# Autodesk Inventor assembly: L22ED01D
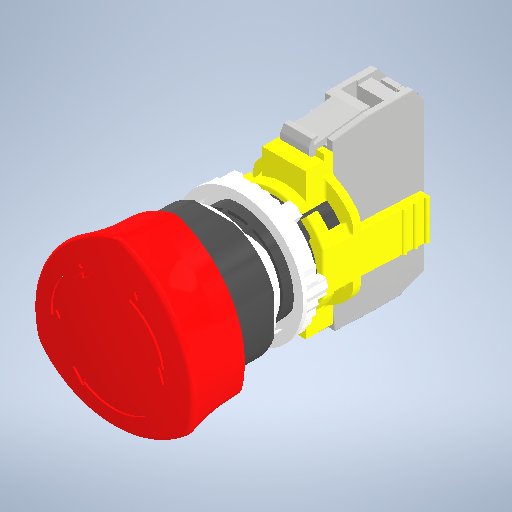
[picture p0: Inventor's stored thumbnail of the model, 512x512]
Saved by Autodesk Inventor 2025.3 (Build 293356000, 356)
## iProperties
Company: Legrand SA
Created: 2008-01-18
Part Number: L22ED01D
Description: STEP AP214
Document SubType Name: Assembly
Designer: louis
Sending System: TRANSCAD
Preprocessor: XStep 1.0
Title: C:/convcao/utilisateur/sortie/fabien.fantini@legrand.fr/21/L22ED01D.stp
## Documents named in this file (19)
- C:\Users\louis\OneDrive\Desktop\R_Trident\02_CAD\01_Standard_Parts\04_ELE_Electrical_Automation\L22ED01D\L22ED01D.iam
- C:\Users\louis\OneDrive\Desktop\R_Trident\02_CAD\01_Standard_Parts\ImportTemp\L22ED01D\L22ED01D\L22ED01D\Part1_Corps principal ( 074228000 - wsp _MASTER -  )_Solide.1 (  de JELE 20955 _ issu de 074228000 - wsp .ipt
- C:\Users\louis\OneDrive\Desktop\R_Trident\02_CAD\01_Standard_Parts\ImportTemp\L22ED01D\L22ED01D\L22ED01D\Part1_Corps de pièce.2 ( _SOL3 - wsp _MASTER -  -Non Smart-  )_Solide.2 (  de JELE 11302 _ issu de _SOL3 .ipt
- C:\Users\louis\OneDrive\Desktop\R_Trident\02_CAD\01_Standard_Parts\ImportTemp\L22ED01D\L22ED01D\L22ED01D\Part1_Corps de pièce.3 ( _SOL4 - wsp _MASTER -  )_Solide.3 (  de JELE 25154 _ issu de _SOL4 - wsp _MASTER.ipt
- C:\Users\louis\OneDrive\Desktop\R_Trident\02_CAD\01_Standard_Parts\ImportTemp\L22ED01D\L22ED01D\L22ED01D\Part1_Corps de pièce.4 ( _SOL5 - wsp _MASTER -  )_Solide.4 (  de JELE 29157 _ issu de _SOL5 - wsp _MASTER.ipt
- C:\Users\louis\OneDrive\Desktop\R_Trident\02_CAD\01_Standard_Parts\ImportTemp\L22ED01D\L22ED01D\L22ED01D\Part1_Corps de pièce.5 ( 075121000 - wsp _MASTER -  )_Solide.5 (  de JELE 40425 _ issu de 075121000 - wsp.ipt
- C:\Users\louis\OneDrive\Desktop\R_Trident\02_CAD\01_Standard_Parts\ImportTemp\L22ED01D\L22ED01D\L22ED01D\Part1_Corps de pièce.6 ( _SOL7 - wsp _MASTER -  )_Solide.6 (  de JELE 41156 _ issu de _SOL7 - wsp _MASTER.ipt
- C:\Users\louis\OneDrive\Desktop\R_Trident\02_CAD\01_Standard_Parts\ImportTemp\L22ED01D\L22ED01D\L22ED01D\Part1_Corps de pièce.7 ( _SOL8 - wsp _MASTER -  )_Solide.7 (  de JELE 64956 _ issu de _SOL8 - wsp _MASTER.ipt
- C:\Users\louis\OneDrive\Desktop\R_Trident\02_CAD\01_Standard_Parts\ImportTemp\L22ED01D\L22ED01D\L22ED01D\Part1_Corps de pièce.8 ( _SOL9 - wsp _MASTER -  -Non Smart-  )_Solide.8 (  de JELE 110028 _ issu de _SOL9.ipt
- C:\Users\louis\OneDrive\Desktop\R_Trident\02_CAD\01_Standard_Parts\ImportTemp\L22ED01D\L22ED01D\L22ED01D\Part1_Corps de pièce.9 ( _SOL10 - wsp _MASTER -  )_Solide.9 (  de JELE 54590 _ issu de _SOL10 - wsp _MAST.ipt
- C:\Users\louis\OneDrive\Desktop\R_Trident\02_CAD\01_Standard_Parts\ImportTemp\L22ED01D\L22ED01D\L22ED01D\Part1_Corps de pièce.10 ( _SOL11 - wsp _MASTER -  -Non Smart-  )_Solide.10 (  de JELE 63513 _ issu de _SO.ipt
- C:\Users\louis\OneDrive\Desktop\R_Trident\02_CAD\01_Standard_Parts\ImportTemp\L22ED01D\L22ED01D\L22ED01D\Part1_Corps de pièce.11 ( _SOL12 - wsp _MASTER -  -Non Smart-  )_Solide.11 (  de JELE 64772 _ issu de _SO.ipt
- C:\Users\louis\OneDrive\Desktop\R_Trident\02_CAD\01_Standard_Parts\ImportTemp\L22ED01D\L22ED01D\L22ED01D\Part1_Corps de pièce.12 ( _SOL13 - wsp _MASTER -  )_Solide.12 (  de JELE 45820 _ issu de _SOL13 - wsp _MA.ipt
- C:\Users\louis\OneDrive\Desktop\R_Trident\02_CAD\01_Standard_Parts\ImportTemp\L22ED01D\L22ED01D\L22ED01D\Part1_Corps de pièce.13 ( _SOL14 - wsp _MASTER -  )_Solide.13 (  de JELE 88964 _ issu de _SOL14 - wsp _MA.ipt
- C:\Users\louis\OneDrive\Desktop\R_Trident\02_CAD\01_Standard_Parts\ImportTemp\L22ED01D\L22ED01D\L22ED01D\Part1_Corps de pièce.14 ( _SOL15 - wsp _MASTER -  )_Solide.14 (  de JELE 108439 _ issu de _SOL15 - wsp _M.ipt
- C:\Users\louis\OneDrive\Desktop\R_Trident\02_CAD\01_Standard_Parts\ImportTemp\L22ED01D\L22ED01D\L22ED01D\Part1_Corps de pièce.15 ( _SOL16 - wsp _MASTER -  -Non Smart-  )_Solide.15 (  de JELE 109844 _ issu de _S.ipt
- C:\Users\louis\OneDrive\Desktop\R_Trident\02_CAD\01_Standard_Parts\ImportTemp\L22ED01D\L22ED01D\L22ED01D\Part1_Corps de pièce.16 ( _SOL17 - wsp _MASTER -  -Non Smart-  )_Solide.16 (  de JELE 110465 _ issu de _S.ipt
- C:\Users\louis\OneDrive\Desktop\R_Trident\02_CAD\01_Standard_Parts\ImportTemp\L22ED01D\L22ED01D\L22ED01D\Part1_Corps de pièce.17 ( _SOL18 - wsp _MASTER -  -Non Smart-  )_Assemble.1.ipt
- C:\Users\louis\OneDrive\Desktop\R_Trident\02_CAD\01_Standard_Parts\ImportTemp\L22ED01D\L22ED01D\L22ED01D\Part1_Corps de pièce.17 ( _SOL18 - wsp _MASTER -  -Non Smart-  )_Assemble.1_1.ipt
## Components (18 placed, 18 different names)
1. Part1_Corps principal ( 074228000 - wsp _MASTER -  )_Solide.1 (  de JELE 20955 _ issu de 074228000 - wsp — Insert:1
2. Part1_Corps de pièce.2 ( _SOL3 - wsp _MASTER -  -Non Smart-  )_Solide.2 (  de JELE 11302 _ issu de _SOL3 — Insert:1
3. Part1_Corps de pièce.3 ( _SOL4 - wsp _MASTER -  )_Solide.3 (  de JELE 25154 _ issu de _SOL4 - wsp _MASTER
4. Part1_Corps de pièce.4 ( _SOL5 - wsp _MASTER -  )_Solide.4 (  de JELE 29157 _ issu de _SOL5 - wsp _MASTER
5. Part1_Corps de pièce.5 ( 075121000 - wsp _MASTER -  )_Solide.5 (  de JELE 40425 _ issu de 075121000 - wsp
6. Part1_Corps de pièce.6 ( _SOL7 - wsp _MASTER -  )_Solide.6 (  de JELE 41156 _ issu de _SOL7 - wsp _MASTER
7. Part1_Corps de pièce.7 ( _SOL8 - wsp _MASTER -  )_Solide.7 (  de JELE 64956 _ issu de _SOL8 - wsp _MASTER
8. Part1_Corps de pièce.8 ( _SOL9 - wsp _MASTER -  -Non Smart-  )_Solide.8 (  de JELE 110028 _ issu de _SOL9
9. Part1_Corps de pièce.9 ( _SOL10 - wsp _MASTER -  )_Solide.9 (  de JELE 54590 _ issu de _SOL10 - wsp _MAST
10. Part1_Corps de pièce.10 ( _SOL11 - wsp _MASTER -  -Non Smart-  )_Solide.10 (  de JELE 63513 _ issu de _SO
11. Part1_Corps de pièce.11 ( _SOL12 - wsp _MASTER -  -Non Smart-  )_Solide.11 (  de JELE 64772 _ issu de _SO
12. Part1_Corps de pièce.12 ( _SOL13 - wsp _MASTER -  )_Solide.12 (  de JELE 45820 _ issu de _SOL13 - wsp _MA
13. Part1_Corps de pièce.13 ( _SOL14 - wsp _MASTER -  )_Solide.13 (  de JELE 88964 _ issu de _SOL14 - wsp _MA
14. Part1_Corps de pièce.14 ( _SOL15 - wsp _MASTER -  )_Solide.14 (  de JELE 108439 _ issu de _SOL15 - wsp _M
15. Part1_Corps de pièce.15 ( _SOL16 - wsp _MASTER -  -Non Smart-  )_Solide.15 (  de JELE 109844 _ issu de _S
16. Part1_Corps de pièce.16 ( _SOL17 - wsp _MASTER -  -Non Smart-  )_Solide.16 (  de JELE 110465 _ issu de _S
17. Part1_Corps de pièce.17 ( _SOL18 - wsp _MASTER -  -Non Smart-  )_Assemble.1
18. Part1_Corps de pièce.17 ( _SOL18 - wsp _MASTER -  -Non Smart-  )_Assemble.1_1
## Relationships (1: Insert 1)
- Insert:1 (1 mm): Part1_Corps principal ( 074228000 - wsp _MASTER -  )_Solide.1 (  de JELE 20955 _ issu de 074228000 - wsp ↔ Part1_Corps de pièce.2 ( _SOL3 - wsp _MASTER -  -Non Smart-  )_Solide.2 (  de JELE 11302 _ issu de _SOL3
